# Autodesk Inventor assembly: RotMotor
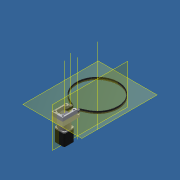
[picture p0: Inventor's stored thumbnail of the model, 180x180]
Saved by Autodesk Inventor 2016 (Build 200138000, 138)
## iProperties
Created: 2015-10-03
Part Number: RotMotor
Material: Generisch
Document SubType Name: Assembly
Designer: 4ndreas
Mass: 1868.19 g
Surface Area: 2604.54 cm^2
Volume: 895.854 cm^3
Density: 2.08538 g/cm^3
Author: 4ndreas
## Documents named in this file (5)
- C:\Users\4ndreas\Documents\github\Mantis-Robot-Arm\MantisRobotArm\Workspace\_assemblys\RotMotor.iam
- C:\Users\4ndreas\Documents\github\Mantis-Robot-Arm\MantisRobotArm\Workspace\_assemblys\RotBase\Konstruktions-Assistent\Übertragung des Zahnriemens1.iam
- C:\Users\4ndreas\Documents\github\Mantis-Robot-Arm\MantisRobotArm\Workspace\_printed parts\RotBase_r1.ipt
- C:\Users\4ndreas\Documents\github\Mantis-Robot-Arm\MantisRobotArm\Workspace\_motors\Nema17_GearedStepper.ipt
- C:\Users\4ndreas\Documents\github\Mantis-Robot-Arm\MantisRobotArm\Workspace\_printed parts\rotMotorMount.ipt
## Components (4 placed, 4 different names)
1. Übertragung des Zahnriemens:1 [sub-assembly] — Passend:7, Passend:11, Passend:12, Passend:16
2. Nema17_GearedStepper:1 — Passend:13, Passend:14, Passend:15
3. RotBase_r1:1 — Passend:6
4. rotMotorMount:1 — Passend:11, Passend:12, Passend:13, Passend:14, Passend:15, Passend:16
## Relationships (8: Mate 8)
- Passend:6 [Mate]: RotBase_r1:1
- Passend:7 [Mate]: Übertragung des Zahnriemens:1
- Passend:11 [Mate]: Übertragung des Zahnriemens:1 ↔ rotMotorMount:1
- Passend:12 [Mate]: Übertragung des Zahnriemens:1 ↔ rotMotorMount:1
- Passend:13 [Mate]: Nema17_GearedStepper:1 ↔ rotMotorMount:1
- Passend:14 [Mate]: Nema17_GearedStepper:1 ↔ rotMotorMount:1
- Passend:15 [Mate]: Nema17_GearedStepper:1 ↔ rotMotorMount:1
- Passend:16 [Mate] (2 mm): Übertragung des Zahnriemens:1 ↔ rotMotorMount:1
